# Autodesk Inventor assembly: Assembly_Cube_Baseplate_4x4_v2
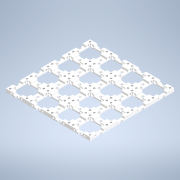
[picture p0: Inventor's stored thumbnail of the model, 180x180]
Saved by Autodesk Inventor 2022 (Build 260153000, 153)
## iProperties
Created: 2021-04-10
Part Number: Assembly_Cube_Baseplate_4x4_v2
Document SubType Name: Assembly
Designer: Hesap
Author: Hesap
## Documents named in this file (2)
- C:\Users\ASUS\Desktop\CAD designs\5. Brewster Angle\Assembly_Cube_Baseplate_4x4_v2.iam
- C:\Users\ASUS\Desktop\CAD designs\1. Crossed Polarizers\Assembly_Cube_Baseplate_4x1_v2.iam
## Components (4 placed, 1 different names)
1. Assembly_Cube_Baseplate_4x1_v2:1 [sub-assembly] — Rotational:2, Rotational:3, Rotational:4, Rotational:5, Rotational:8, Rotational:9
2. Assembly_Cube_Baseplate_4x1_v2:2 [sub-assembly] — Rotational:4, Rotational:5, Rotational:7, Rotational:8, Rotational:9
3. Assembly_Cube_Baseplate_4x1_v2:3 [sub-assembly] — Rotational:1, Rotational:6
4. Assembly_Cube_Baseplate_4x1_v2:4 [sub-assembly] — Rotational:1, Rotational:2, Rotational:3, Rotational:6, Rotational:7
## Relationships (9: RevoluteJoint 9)
- Rotational:1 [RevoluteJoint]: Assembly_Cube_Baseplate_4x1_v2:3 ↔ Assembly_Cube_Baseplate_4x1_v2:4
- Rotational:2 [RevoluteJoint]: Assembly_Cube_Baseplate_4x1_v2:1 ↔ Assembly_Cube_Baseplate_4x1_v2:4
- Rotational:3 [RevoluteJoint]: Assembly_Cube_Baseplate_4x1_v2:1 ↔ Assembly_Cube_Baseplate_4x1_v2:4
- Rotational:4 [RevoluteJoint]: Assembly_Cube_Baseplate_4x1_v2:1 ↔ Assembly_Cube_Baseplate_4x1_v2:2
- Rotational:5 [RevoluteJoint]: Assembly_Cube_Baseplate_4x1_v2:1 ↔ Assembly_Cube_Baseplate_4x1_v2:2
- Rotational:6 [RevoluteJoint]: Assembly_Cube_Baseplate_4x1_v2:3 ↔ Assembly_Cube_Baseplate_4x1_v2:4
- Rotational:7 [RevoluteJoint]: Assembly_Cube_Baseplate_4x1_v2:2 ↔ Assembly_Cube_Baseplate_4x1_v2:4
- Rotational:8 [RevoluteJoint]: Assembly_Cube_Baseplate_4x1_v2:1 ↔ Assembly_Cube_Baseplate_4x1_v2:2
- Rotational:9 [RevoluteJoint]: Assembly_Cube_Baseplate_4x1_v2:1 ↔ Assembly_Cube_Baseplate_4x1_v2:2
